# Autodesk Inventor assembly: ManganPitik
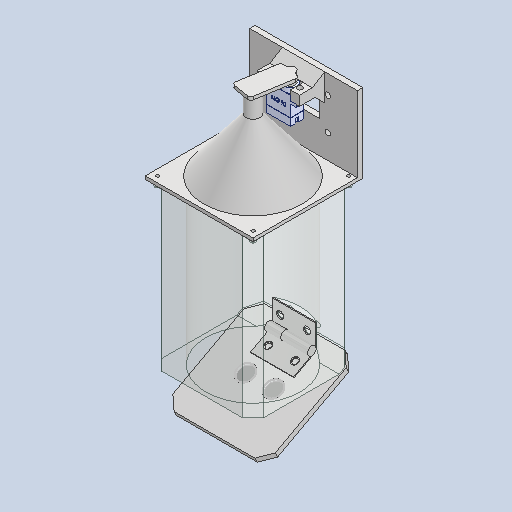
[picture p0: Inventor's stored thumbnail of the model, 512x512]
Saved by Autodesk Inventor 2026.2 (Build 302298010, 298A)
## iProperties
Created: 2026-05-22
Part Number: ManganPitik
Document SubType Name: Assembly
Designer: rizky
Author: rizky
## Documents named in this file (9)
- C:\SEMESTER 4\Mikrokontroller\PakanPitik\3D Design\ManganPitik.iam
- C:\SEMESTER 4\TEKNOFEST\Robolig\GripperGeser\servo-motor-sg90-mg90-1.snapshot.9\mg 90 micro servo\mg 90 micro servo\mg 90 micro servo.ipt
- C:\SEMESTER 4\Mikrokontroller\PakanPitik\3D Design\TutupTank.ipt
- C:\SEMESTER 4\Mikrokontroller\PakanPitik\3D Design\CorongBawah.ipt
- C:\SEMESTER 4\Mikrokontroller\PakanPitik\3D Design\Tank.ipt
- C:\SEMESTER 4\Mikrokontroller\PakanPitik\3D Design\TutupAtas.ipt
- C:\Users\rizky\Downloads\hcsr-04-ultrasonic-sensor-1.snapshot.1\Ultrasonic HC-SR04\Ultrasonic HC-SR04\Ultrasonic HC-SR04.ipt
- C:\Users\rizky\Downloads\hinges-1-1-2-inches-1.snapshot.4\Engsel 1 inch setengah\Engsel Female.ipt
- C:\Users\rizky\Downloads\hinges-1-1-2-inches-1.snapshot.4\Engsel 1 inch setengah\Engsel Male.ipt
## Components (8 placed, 8 different names)
1. mg 90 micro servo:1 — Mate:5, Mate:6, Mate:7, Mate:8, Mate:9
2. CorongBawah:1 — Mate:5, Mate:8, Mate:9, Mate:10, Mate:11, Mate:12
3. TutupTank:1 — Mate:6, Mate:7
4. Tank:1 — Mate:10, Mate:11, Mate:12, Mate:41, Mate:42, Mate:43
5. TutupAtas:1 — Mate:31, Mate:34, Mate:38, Mate:44, Mate:45, Mate:46
6. Ultrasonic HC-SR04:1 — Mate:31, Mate:34, Mate:38
7. Engsel Female:1 — Mate:39, Mate:40, Mate:44, Mate:45, Mate:46
8. Engsel Male:1 — Mate:39, Mate:40, Mate:41, Mate:42, Mate:43
## Relationships (19: Mate 19)
- Mate:5: mg 90 micro servo:1 ↔ CorongBawah:1
- Mate:6: mg 90 micro servo:1 ↔ TutupTank:1
- Mate:7: mg 90 micro servo:1 ↔ TutupTank:1
- Mate:8: mg 90 micro servo:1 ↔ CorongBawah:1
- Mate:9: mg 90 micro servo:1 ↔ CorongBawah:1
- Mate:10: CorongBawah:1 ↔ Tank:1
- Mate:11: CorongBawah:1 ↔ Tank:1
- Mate:12: CorongBawah:1 ↔ Tank:1
- Mate:31: TutupAtas:1 ↔ Ultrasonic HC-SR04:1
- Mate:34: TutupAtas:1 ↔ Ultrasonic HC-SR04:1
- Mate:38: TutupAtas:1 ↔ Ultrasonic HC-SR04:1
- Mate:39: Engsel Female:1 ↔ Engsel Male:1
- Mate:40: Engsel Female:1 ↔ Engsel Male:1
- Mate:41: Tank:1 ↔ Engsel Male:1
- Mate:42: Tank:1 ↔ Engsel Male:1
- Mate:43: Tank:1 ↔ Engsel Male:1
- Mate:44: TutupAtas:1 ↔ Engsel Female:1
- Mate:45: TutupAtas:1 ↔ Engsel Female:1
- Mate:46: TutupAtas:1 ↔ Engsel Female:1
